# Autodesk Inventor assembly: claws_endeffector_8_2
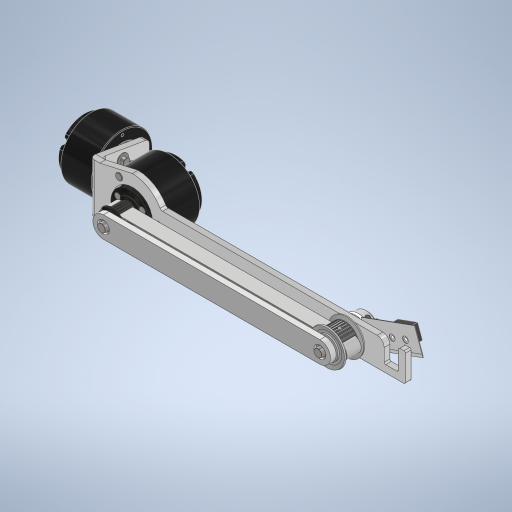
[picture p0: Inventor's stored thumbnail of the model, 512x512]
Saved by Autodesk Inventor 2024 (Build 280153000, 153)
## iProperties
Created: 2025-05-25
Part Number: claws_endeffector_8_2
Document SubType Name: Assembly
Designer: 1412z
Author: 1412z
## Documents named in this file (20)
- C:\Users\1412z\OneDrive\デスクトップ\rdclab\harvesting_robot\harvesting_endeffector\claws_endeffector\claws_endeffector_8_2.iam
- C:\Users\1412z\OneDrive\デスクトップ\rdclab\harvesting_robot\harvesting_endeffector\claws_endeffector\motor_holder\motor_holder_8-2.ipt
- C:\Users\1412z\OneDrive\デスクトップ\rdclab\harvesting_robot\harvesting_endeffector\claws_endeffector\GIM3505-08\GIM3505-8_with-driver.ipt
- C:\Users\1412z\OneDrive\デスクトップ\rdclab\harvesting_robot\harvesting_endeffector\claws_endeffector\misumi\SFL674ZZ_Autodesk_Inventor_2024_20250304\SFL674ZZ.ipt
- C:\Users\1412z\OneDrive\デスクトップ\rdclab\harvesting_robot\harvesting_endeffector\claws_endeffector\misumi\simring\simring_Φ4-Φ5.ipt
- C:\Users\1412z\OneDrive\デスクトップ\rdclab\harvesting_robot\harvesting_endeffector\claws_endeffector\misumi\HTPA32S2M100-A-P4_Autodesk_Inventor_2024_20250404\AIS2024\HTPA32S2M100-A-P4.iam
- C:\Users\1412z\OneDrive\デスクトップ\rdclab\harvesting_robot\harvesting_endeffector\claws_endeffector\misumi\HTPA22S2M100-A-V4-Z6-J3_Autodesk_Inventor_2024_20250304\HTPA22S2M100-A-V4-Z6-J3_0_a-3.ipt
- C:\Users\1412z\OneDrive\デスクトップ\rdclab\harvesting_robot\harvesting_endeffector\claws_endeffector\misumi\M2.5×4\M2.5×4.ipt
- C:\Users\1412z\OneDrive\デスクトップ\rdclab\harvesting_robot\harvesting_endeffector\claws_endeffector\misumi\washer\washer_M3.ipt
- C:\Users\1412z\OneDrive\デスクトップ\rdclab\harvesting_robot\harvesting_endeffector\claws_endeffector\misumi\washer\washer_M4.ipt
- C:\Users\1412z\OneDrive\デスクトップ\rdclab\harvesting_robot\harvesting_endeffector\claws_endeffector\motor_holder\motor_holder_top_2.ipt
- C:\Users\1412z\OneDrive\デスクトップ\rdclab\harvesting_robot\harvesting_endeffector\claws_endeffector\cutter_part\cutter_board_claws_endeffector_8.ipt
- C:\Users\1412z\OneDrive\デスクトップ\rdclab\harvesting_robot\harvesting_endeffector\claws_endeffector\misumi\SSCMN4_Autodesk_Inventor_2024_20250310\AIS2024\SSCMN4.iam
- C:\Users\1412z\OneDrive\デスクトップ\rdclab\harvesting_robot\harvesting_endeffector\claws_endeffector\misumi\M3×8\M3×8.ipt
- C:\Users\1412z\OneDrive\デスクトップ\rdclab\harvesting_robot\harvesting_endeffector\claws_endeffector\misumi\shaft\shaft_15.05.ipt
- C:\Users\1412z\OneDrive\デスクトップ\rdclab\harvesting_robot\harvesting_endeffector\claws_endeffector\misumi\shaft\shaft_31.3mm.ipt
- C:\Users\1412z\OneDrive\デスクトップ\rdclab\harvesting_robot\harvesting_endeffector\claws_endeffector\misumi\M3×4\M3×4.ipt
- C:\Users\1412z\OneDrive\デスクトップ\rdclab\harvesting_robot\harvesting_endeffector\claws_endeffector\misumi\HTBN360S2M-100_Autodesk_Inventor_2024_20250304\HTBN360S2M-100_info-1-16-16.ipt
- C:\Users\1412z\OneDrive\デスクトップ\rdclab\harvesting_robot\harvesting_endeffector\claws_endeffector\cutter_part\cutter_XB210.ipt
- C:\Users\1412z\OneDrive\デスクトップ\rdclab\harvesting_robot\harvesting_endeffector\claws_endeffector\cutter_part\nitrile_rubber.ipt
## Components (39 placed, 19 different names)
1. motor_holder_8-2:1 — 回転:1, 回転:2, 回転:3, 回転:4, 回転:5, 回転:6, 回転:12, 回転:13, 回転:14, 回転:18, 回転:19, 回転:20
2. GIM3505-8_with-driver:1 — 回転:1, 回転:2, 回転:10, 回転:11
3. GIM3505-8_with-driver:2 — 回転:3, 回転:4
4. SFL674ZZ:1 — 回転:5, 回転:8
5. SFL674ZZ:2 — 回転:6, 回転:7
6. simring_Φ4-Φ5:1 — 回転:8, 回転:29
7. simring_Φ4-Φ5:2 — 回転:7, 回転:9
8. HTPA32S2M100-A-P4:1 [sub-assembly] — 回転:9, リジッド:1
9. HTPA22S2M100-A-V4-Z6-J3_0_a-3:1 — 回転:10, 回転:11, 回転:15, 回転:16, 回転:17, 回転:24, 回転:35, 回転:37
10. M2.5×4:1 — 回転:17
11. M2.5×4:2 — 回転:16
12. M2.5×4:3 — 回転:15
13. M2.5×4:4 — 回転:14
14. M2.5×4:5 — 回転:13
15. M2.5×4:6 — 回転:12
16. washer_M3:1 — 回転:20, 回転:23
17. washer_M3:2 — 回転:19, 回転:22
18. washer_M3:3 — 回転:18, 回転:21
19. M2.5×4:7 — 回転:23
20. M2.5×4:8 — 回転:22
21. M2.5×4:9 — 回転:21
22. washer_M4:1 — リジッド:1, 回転:25
23. washer_M4:2 — 回転:24, 回転:26
24. motor_holder_top_2:1 — 回転:25, 回転:26, 回転:27, 回転:28
25. SFL674ZZ:3 — 回転:27, 回転:34
26. SFL674ZZ:4 — 回転:28
27. cutter_board_claws_endeffector_8:1 — 回転:29, 回転:30, 回転:31, 回転:40, 回転:41, スライダ:1
28. SSCMN4:1 [sub-assembly] — 回転:30, 回転:31, 回転:32, 回転:33
29. M3×8:1 — 回転:32
30. M3×8:2 — 回転:33
31. shaft_15.05:1 — 回転:37, 回転:39
32. shaft_31.3mm:1 — 回転:34, 回転:38
33. washer_M3:4 — 回転:35, 回転:36
34. M3×8:3 — 回転:36
35. M3×4:1 — 回転:39
36. M3×4:2 — 回転:38
37. HTBN360S2M-100_info-1-16-16:1
38. cutter_XB210:1 — 回転:40, 回転:41
39. nitrile_rubber:1 — スライダ:1
## Relationships (43: RevoluteJoint 41, WeldJoint 1, TranslationJoint 1)
- 回転:1 [RevoluteJoint]: motor_holder_8-2:1 ↔ GIM3505-8_with-driver:1
- 回転:2 [RevoluteJoint]: motor_holder_8-2:1 ↔ GIM3505-8_with-driver:1
- 回転:3 [RevoluteJoint]: motor_holder_8-2:1 ↔ GIM3505-8_with-driver:2
- 回転:4 [RevoluteJoint]: motor_holder_8-2:1 ↔ GIM3505-8_with-driver:2
- 回転:5 [RevoluteJoint]: motor_holder_8-2:1 ↔ SFL674ZZ:1
- 回転:6 [RevoluteJoint]: motor_holder_8-2:1 ↔ SFL674ZZ:2
- 回転:7 [RevoluteJoint]: SFL674ZZ:2 ↔ simring_Φ4-Φ5:2
- 回転:8 [RevoluteJoint]: SFL674ZZ:1 ↔ simring_Φ4-Φ5:1
- 回転:9 [RevoluteJoint]: simring_Φ4-Φ5:2 ↔ HTPA32S2M100-A-P4:1
- 回転:10 [RevoluteJoint]: GIM3505-8_with-driver:1 ↔ HTPA22S2M100-A-V4-Z6-J3_0_a-3:1
- 回転:11 [RevoluteJoint]: GIM3505-8_with-driver:1 ↔ HTPA22S2M100-A-V4-Z6-J3_0_a-3:1
- 回転:12 [RevoluteJoint]: motor_holder_8-2:1 ↔ M2.5×4:6
- 回転:13 [RevoluteJoint]: motor_holder_8-2:1 ↔ M2.5×4:5
- 回転:14 [RevoluteJoint]: motor_holder_8-2:1 ↔ M2.5×4:4
- 回転:15 [RevoluteJoint]: HTPA22S2M100-A-V4-Z6-J3_0_a-3:1 ↔ M2.5×4:3
- 回転:16 [RevoluteJoint]: HTPA22S2M100-A-V4-Z6-J3_0_a-3:1 ↔ M2.5×4:2
- 回転:17 [RevoluteJoint]: HTPA22S2M100-A-V4-Z6-J3_0_a-3:1 ↔ M2.5×4:1
- 回転:18 [RevoluteJoint]: motor_holder_8-2:1 ↔ washer_M3:3
- 回転:19 [RevoluteJoint]: motor_holder_8-2:1 ↔ washer_M3:2
- 回転:20 [RevoluteJoint]: motor_holder_8-2:1 ↔ washer_M3:1
- 回転:21 [RevoluteJoint]: washer_M3:3 ↔ M2.5×4:9
- 回転:22 [RevoluteJoint]: washer_M3:2 ↔ M2.5×4:8
- 回転:23 [RevoluteJoint]: washer_M3:1 ↔ M2.5×4:7
- 回転:24 [RevoluteJoint]: HTPA22S2M100-A-V4-Z6-J3_0_a-3:1 ↔ washer_M4:2
- リジッド:1 [WeldJoint]: HTPA32S2M100-A-P4:1 ↔ washer_M4:1
- 回転:25 [RevoluteJoint]: washer_M4:1 ↔ motor_holder_top_2:1
- 回転:26 [RevoluteJoint]: washer_M4:2 ↔ motor_holder_top_2:1
- 回転:27 [RevoluteJoint]: motor_holder_top_2:1 ↔ SFL674ZZ:3
- 回転:28 [RevoluteJoint]: motor_holder_top_2:1 ↔ SFL674ZZ:4
- 回転:29 [RevoluteJoint]: simring_Φ4-Φ5:1 ↔ cutter_board_claws_endeffector_8:1
- 回転:30 [RevoluteJoint]: cutter_board_claws_endeffector_8:1 ↔ SSCMN4:1
- 回転:31 [RevoluteJoint]: cutter_board_claws_endeffector_8:1 ↔ SSCMN4:1
- 回転:32 [RevoluteJoint]: SSCMN4:1 ↔ M3×8:1
- 回転:33 [RevoluteJoint]: SSCMN4:1 ↔ M3×8:2
- 回転:34 [RevoluteJoint]: SFL674ZZ:3 ↔ shaft_31.3mm:1
- 回転:35 [RevoluteJoint]: HTPA22S2M100-A-V4-Z6-J3_0_a-3:1 ↔ washer_M3:4
- 回転:36 [RevoluteJoint]: washer_M3:4 ↔ M3×8:3
- 回転:37 [RevoluteJoint]: HTPA22S2M100-A-V4-Z6-J3_0_a-3:1 ↔ shaft_15.05:1
- 回転:38 [RevoluteJoint]: shaft_31.3mm:1 ↔ M3×4:2
- 回転:39 [RevoluteJoint]: shaft_15.05:1 ↔ M3×4:1
- 回転:40 [RevoluteJoint]: cutter_board_claws_endeffector_8:1 ↔ cutter_XB210:1
- 回転:41 [RevoluteJoint]: cutter_board_claws_endeffector_8:1 ↔ cutter_XB210:1
- スライダ:1 [TranslationJoint]: cutter_board_claws_endeffector_8:1 ↔ nitrile_rubber:1
